# Autodesk Inventor assembly: RobotMechanika
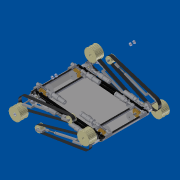
[picture p0: Inventor's stored thumbnail of the model, 180x180]
Saved by Autodesk Inventor 2015 SP1 (Build 190203100, 203)
## iProperties
Created: 2014-09-09
Part Number: RobotMechanika
Document SubType Name: Assembly
Designer: laca
Mass: 3656.47 g
Surface Area: 16588.1 cm^2
Volume: 1645.24 cm^3
Density: 2.22245 g/cm^3
Author: laca
## Documents named in this file (3)
- C:\Users\laca\Desktop\RobotMechanika\RobotMechanika.iam
- C:\Users\laca\Desktop\RobotMechanika\FelAlvaz.iam
- C:\Users\laca\Desktop\RobotMechanika\Lemez.ipt
## Components (3 placed, 2 different names)
1. FelAlvaz:1 [sub-assembly] — Rigid:1
2. FelAlvaz:2 [sub-assembly] — Rigid:1, Flush:1, Mate:1, Mate:2
3. Lemez:1 — Flush:1, Mate:1, Mate:2
## Relationships (4: Mate 2, WeldJoint 1, Flush 1)
- Rigid:1 [WeldJoint]: FelAlvaz:1 ↔ FelAlvaz:2
- Flush:1: FelAlvaz:2 ↔ Lemez:1
- Mate:1: FelAlvaz:2 ↔ Lemez:1
- Mate:2: FelAlvaz:2 ↔ Lemez:1
